# Autodesk Inventor assembly: assembly
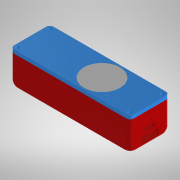
[picture p0: Inventor's stored thumbnail of the model, 180x180]
Saved by Autodesk Inventor 2022 (Build 260153000, 153)
## iProperties
Created: 2024-12-05
Part Number: assembly
Document SubType Name: Assembly
Designer: seama
Author: seama
## Documents named in this file (5)
- D:\devlopment\TVOCMeter\parts\assembly.iam
- D:\devlopment\TVOCMeter\parts\case_front.ipt
- D:\devlopment\TVOCMeter\parts\oled_display_fixer.ipt
- D:\devlopment\TVOCMeter\parts\case_back.ipt
- D:\devlopment\TVOCMeter\parts\vent_hole_cover.ipt
## Components (4 placed, 4 different names)
1. case_front:1 — 플러쉬:1, 플러쉬:2, 플러쉬:3, 회전:1
2. oled_display_fixer:1 — 회전:1
3. case_back:1 — 플러쉬:1, 플러쉬:2, 플러쉬:3, 삽입:1
4. vent_hole_cover:1 — 삽입:1
## Relationships (5: Flush 3, RevoluteJoint 1, Insert 1)
- 플러쉬:1 [Flush] (-3 mm): case_front:1 ↔ case_back:1
- 플러쉬:2 [Flush]: case_front:1 ↔ case_back:1
- 플러쉬:3 [Flush]: case_front:1 ↔ case_back:1
- 회전:1 [RevoluteJoint] (-1.2 mm): case_front:1 ↔ oled_display_fixer:1
- 삽입:1 [Insert]: case_back:1 ↔ vent_hole_cover:1
